# Autodesk Inventor assembly: Z Drive B
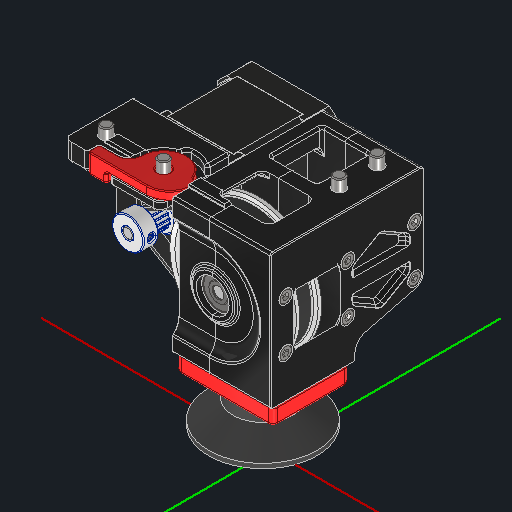
[picture p0: Inventor's stored thumbnail of the model, 512x512]
Saved by Autodesk Inventor 2022.2 (Build 262287010, 287A)
## iProperties
Created: 2022-03-12
Part Number: Z Drive B
Document SubType Name: Assembly
Designer: sleib
Author: sleib
## Documents named in this file (4)
- C:\Users\sleib\Projekte\Voron-2\CAD\Inventor\Z Drive [B].iam
- C:\Users\sleib\Projekte\Voron-2\CAD\Inventor\Z Belt-Drive Unit [B].iam
- C:\Users\sleib\Projekte\Voron-2\CAD\Inventor\Z Motor-Unit [B].iam
- C:\Users\sleib\Projekte\Voron-2\CAD\Inventor\GT2 188mm Belt Loop.ipt
## Components (3 placed, 3 different names)
1. Z Belt-Drive Unit [B]:1 [sub-assembly] — Passend:1, Passend:2, Fluchtend:1
2. Z Motor-Unit [B]:1 [sub-assembly] — Passend:3, Passend:4, Fluchtend:1
3. GT2 188mm Belt Loop:1 — Passend:1, Passend:2, Passend:3, Passend:4
## Relationships (5: Mate 4, Flush 1)
- Passend:1 [Mate]: Z Belt-Drive Unit [B]:1 ↔ GT2 188mm Belt Loop:1
- Passend:2 [Mate] (0.5 mm): Z Belt-Drive Unit [B]:1 ↔ GT2 188mm Belt Loop:1
- Passend:3 [Mate]: Z Motor-Unit [B]:1 ↔ GT2 188mm Belt Loop:1
- Passend:4 [Mate] (0.5 mm): Z Motor-Unit [B]:1 ↔ GT2 188mm Belt Loop:1
- Fluchtend:1 [Flush]: Z Belt-Drive Unit [B]:1 ↔ Z Motor-Unit [B]:1
